# Autodesk Inventor assembly: mobile_robot
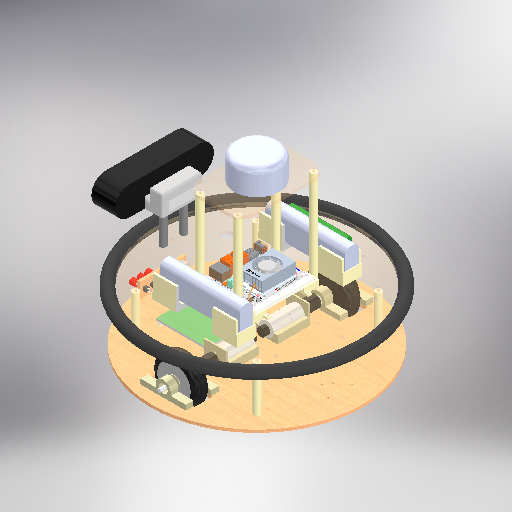
[picture p0: Inventor's stored thumbnail of the model, 512x512]
Saved by Autodesk Inventor 2026 (Build 300175050, 175E)
## iProperties
Created: 2025-06-04
Part Number: mobile_robot
Document SubType Name: Assembly
Designer: satom
Author: satom
## Documents named in this file (32)
- C:\Users\satom\Desktop\Robot\CAD\Inventor\mobile_robot_short.iam
- C:\Users\satom\Desktop\Robot\CAD\Inventor\C - Chassis\layer1.ipt
- C:\Users\satom\Desktop\Robot\CAD\Inventor\D - DriveTrain\wheel_bearing.ipt
- C:\Users\satom\Desktop\Robot\CAD\Inventor\D - DriveTrain\wheel_mount.ipt
- C:\Users\satom\Desktop\Robot\CAD\Inventor\D - DriveTrain\motor_holder.ipt
- C:\Users\satom\Desktop\Robot\CAD\Inventor\solidworks\D - DriveTrain\ball_caster\ball_caster\ball_caster.ipt
- C:\Users\satom\Desktop\Robot\CAD\Inventor\solidworks\D - DriveTrain\motor\motor\motor.ipt
- C:\Users\satom\Desktop\Robot\CAD\Inventor\solidworks\D - DriveTrain\wheel\wheel\wheel.ipt
- C:\Users\satom\Desktop\Robot\CAD\Inventor\solidworks\D - DriveTrain\drive_shaft\drive_shaft\drive_shaft.ipt
- C:\Users\satom\Desktop\Robot\CAD\Inventor\solidworks\D - DriveTrain\ball_bearing\ball_bearing\ball_bearing.ipt
- C:\Users\satom\Desktop\Robot\CAD\Inventor\solidworks\D - DriveTrain\shaft_coupler 6 mm\shaft_coupler 6 mm\shaft_coupler 6 mm.ipt
- C:\Users\satom\Desktop\Robot\CAD\Inventor\solidworks\E - Electronics\Main Board\Main Board\Main Board.ipt
- C:\Users\satom\Desktop\Robot\CAD\Inventor\E - Electronics\1-4_inch_standoff.ipt
- C:\Users\satom\Desktop\Robot\CAD\Inventor\C - Chassis\3inch_standoff.ipt
- C:\Users\satom\Desktop\Robot\CAD\Inventor\C - Chassis\control_panel.ipt
- C:\Users\satom\Desktop\Robot\CAD\Inventor\E - Electronics\status_LED\status_LED\status_LED.ipt
- C:\Users\satom\Desktop\Robot\CAD\Inventor\E - Electronics\rocker_switch\rocker_switch\rocker_switch.ipt
- C:\Users\satom\Desktop\Robot\CAD\Inventor\E - Electronics\button\button\button.ipt
- C:\Users\satom\Desktop\Robot\CAD\Inventor\solidworks\E - Electronics\NiMH_battery\NiMH_battery\NiMH_battery.ipt
- C:\Users\satom\Desktop\Robot\CAD\Inventor\E - Electronics\NiMH_Holder_Front.ipt
- C:\Users\satom\Desktop\Robot\CAD\Inventor\E - Electronics\NiMH_Holder_Back.ipt
- C:\Users\satom\Desktop\Robot\CAD\Inventor\solidworks\E - Electronics\Lion_5V\Lion_5V\Lion_5V.ipt
- C:\Users\satom\Desktop\Robot\CAD\Inventor\E - Electronics\jetson_orin_nano_holder_corner_1.ipt
- C:\Users\satom\Desktop\Robot\CAD\Inventor\E - Electronics\jetson_orin_nano_holder_corner_2.ipt
- C:\Users\satom\Desktop\Robot\CAD\Inventor\E - Electronics\orin_nano\orin_nano\orin_nano.ipt
- C:\Users\satom\Desktop\Robot\CAD\Inventor\C - Chassis\layer2_short.ipt
- C:\Users\satom\Desktop\Robot\CAD\Inventor\C - Chassis\foam_bumper_circular.ipt
- C:\Users\satom\Desktop\Robot\CAD\Inventor\C - Chassis\LiDAR_plate.ipt
- C:\Users\satom\Desktop\Robot\CAD\Inventor\E - Electronics\astra_camera.ipt
- C:\Users\satom\Desktop\Robot\CAD\Inventor\E - Electronics\astra_holder.ipt
- C:\Users\satom\Desktop\Robot\CAD\Inventor\solidworks\E - Electronics\A2_LIDAR\A2_LIDAR\A2_LIDAR.ipt
- C:\Users\satom\Desktop\Robot\CAD\Inventor\C - Chassis\6inch_standoff.ipt
## Components (62 placed, 31 different names)
1. layer1:1 — Mate:1, Mate:2, Mate:3, Mate:4, Mate:5, Mate:6, Mate:7, Mate:8, Mate:9, Mate:10, Mate:11, Mate:12, Mate:13, Mate:14, Mate:15, Mate:16, Mate:17, Mate:18, Mate:19, Mate:20, Mate:21, Mate:22, Mate:23, Mate:56, Mate:57, Mate:66, Mate:67, Mate:68, Mate:69, Mate:70, Mate:71, Mate:72, Mate:73, Mate:74, Mate:75, Mate:76, Flush:3, Mate:88, Mate:89
2. wheel_bearing:1 — Mate:7, Mate:8, Mate:16, Mate:40, Mate:41
3. wheel_mount:1 — Mate:32, Mate:33, Flush:2
4. motor_holder:1 — Mate:2, Mate:3, Mate:26, Mate:27, Mate:56, Mate:57
5. wheel_bearing:2 — Mate:9, Mate:10, Mate:14, Mate:15, Mate:46, Mate:47
6. wheel_mount:2 — Mate:28, Mate:29, Flush:1, Mate:36, Mate:37
7. motor_holder:2 — Mate:1, Mate:4, Mate:24, Mate:25
8. wheel_bearing:3 — Mate:11, Mate:12, Mate:13, Mate:44, Mate:45
9. wheel_mount:3 — Mate:30, Mate:31, Flush:1
10. wheel_bearing:4 — Mate:5, Mate:6, Mate:17, Mate:42, Mate:43
11. wheel_mount:4 — Mate:34, Mate:35, Flush:2, Mate:38, Mate:39
12. ball_caster:1 — Mate:19, Mate:22, Mate:23
13. ball_caster:2 — Mate:18, Mate:20, Mate:21
14. motor:1 — Mate:24, Mate:25, Mate:48, Mate:51
15. motor:2 — Mate:26, Mate:27, Mate:52, Mate:55
16. wheel:1 — Mate:32, Mate:33, Mate:34, Mate:35
17. wheel:2 — Mate:28, Mate:29, Mate:30, Mate:31
18. drive_shaft:1 — Mate:38, Mate:39, Mate:49, Mate:50
19. drive_shaft:2 — Mate:36, Mate:37, Mate:53, Mate:54
20. ball_bearing:1 — Mate:42, Mate:43
21. ball_bearing:2 — Mate:40, Mate:41
22. ball_bearing:3 — Mate:44, Mate:45, Mate:49
23. ball_bearing:4 — Mate:46, Mate:47
24. shaft_coupler 6 mm:1 — Mate:48, Mate:50, Mate:51
25. shaft_coupler 6 mm:2 — Mate:52, Mate:53, Mate:54, Mate:55
26. Main Board:1 — Mate:61, Mate:62, Mate:63, Mate:64, Mate:65
27. 1-4_inch_standoff:1 — Mate:62, Mate:65
28. 1-4_inch_standoff:2 — Mate:63, Mate:64, Mate:66, Mate:67
29. 1-4_inch_standoff:3 — Mate:61, Mate:68
30. 1-4_inch_standoff:4
31. 3inch_standoff:1 — Mate:69, Mate:71
32. 3inch_standoff:2 — Mate:70, Mate:72, Mate:132
33. 3inch_standoff:3 — Mate:73, Mate:74
34. 3inch_standoff:4 — Mate:75, Mate:76, Mate:130, Mate:131
35. control_panel:1 — Flush:3, Mate:88, Mate:89
36. status_LED:1
37. rocker_switch:1
38. button:1
39. button:2
40. button:3
41. NiMH_battery:1 — Mate:135
42. NiMH_battery:2 — Mate:147
43. NiMH_Holder_Front:1 — Mate:134, Mate:138, Mate:139
44. NiMH_Holder_Back:1 — Mate:133, Mate:135, Mate:136, Mate:137
45. NiMH_Holder_Back:2 — Mate:141, Mate:142, Mate:143, Mate:147
46. NiMH_Holder_Front:2 — Mate:144, Mate:145, Mate:146, Mate:148, Flush:151
47. Lion_5V:1 — Mate:148, Flush:151, Mate:149
48. jetson_orin_nano_holder_corner_1:1 — Mate:154, Mate:155
49. jetson_orin_nano_holder_corner_1:2 — Mate:129, Mate:150, Mate:151
50. jetson_orin_nano_holder_corner_2:1 — Mate:156, Mate:157
51. jetson_orin_nano_holder_corner_2:2 — Mate:152, Mate:153
52. orin_nano:1 — Mate:129
53. layer2_short:1 — Mate:130, Mate:131, Mate:132, Mate:133, Mate:134, Mate:136, Mate:137, Mate:138, Mate:139, Mate:141, Mate:142, Mate:143, Mate:144, Mate:145, Mate:146, Mate:149, Mate:150, Mate:151, Mate:152, Mate:153, Mate:154, Mate:155, Mate:156, Mate:157, Mate:158, Mate:159, Mate:164, Mate:165, Mate:166, Mate:168, Mate:169, Mate:170, Mate:171, Mate:178, Mate:179
54. foam_bumper_circular:1 — Mate:158, Mate:159
55. LiDAR_plate:1 — Mate:160, Mate:161, Mate:162, Mate:172, Mate:173, Mate:174, Mate:175, Mate:176, Mate:177
56. astra_camera:1 — Mate:163, Flush:152, Mate:167
57. astra_holder:1 — Mate:163, Mate:164, Mate:165, Mate:166, Flush:152, Mate:167
58. A2_LIDAR:1 — Mate:160, Mate:161, Mate:162
59. 6inch_standoff:1 — Mate:171, Mate:176
60. 6inch_standoff:2 — Mate:168, Mate:174, Mate:175, Mate:179
61. 6inch_standoff:3 — Mate:169, Mate:177, Mate:178
62. 6inch_standoff:4 — Mate:170, Mate:172, Mate:173
## Relationships (149: Mate 144, Flush 5)
- Mate:1: layer1:1 ↔ motor_holder:2
- Mate:2: layer1:1 ↔ motor_holder:1
- Mate:3: layer1:1 ↔ motor_holder:1
- Mate:4: layer1:1 ↔ motor_holder:2
- Mate:5: layer1:1 ↔ wheel_bearing:4
- Mate:6: layer1:1 ↔ wheel_bearing:4
- Mate:7: layer1:1 ↔ wheel_bearing:1
- Mate:8: layer1:1 ↔ wheel_bearing:1
- Mate:9: layer1:1 ↔ wheel_bearing:2
- Mate:10: layer1:1 ↔ wheel_bearing:2
- Mate:11: layer1:1 ↔ wheel_bearing:3
- Mate:12: layer1:1 ↔ wheel_bearing:3
- Mate:13: layer1:1 ↔ wheel_bearing:3
- Mate:14: layer1:1 ↔ wheel_bearing:2
- Mate:15: layer1:1 ↔ wheel_bearing:2
- Mate:16: layer1:1 ↔ wheel_bearing:1
- Mate:17: layer1:1 ↔ wheel_bearing:4
- Mate:18: layer1:1 ↔ ball_caster:2
- Mate:19: layer1:1 ↔ ball_caster:1
- Mate:20: layer1:1 ↔ ball_caster:2
- Mate:21: layer1:1 ↔ ball_caster:2
- Mate:22: layer1:1 ↔ ball_caster:1
- Mate:23: layer1:1 ↔ ball_caster:1
- Mate:24: motor_holder:2 ↔ motor:1
- Mate:25: motor_holder:2 ↔ motor:1
- Mate:26: motor_holder:1 ↔ motor:2
- Mate:27: motor_holder:1 ↔ motor:2
- Mate:28: wheel_mount:2 ↔ wheel:2
- Mate:29: wheel_mount:2 ↔ wheel:2
- Mate:30: wheel_mount:3 ↔ wheel:2
- Mate:31: wheel_mount:3 ↔ wheel:2
- Flush:1: wheel_mount:2 ↔ wheel_mount:3
- Mate:32: wheel_mount:1 ↔ wheel:1
- Mate:33: wheel_mount:1 ↔ wheel:1
- Mate:34: wheel_mount:4 ↔ wheel:1
- Mate:35: wheel_mount:4 ↔ wheel:1
- Flush:2: wheel_mount:1 ↔ wheel_mount:4
- Mate:36: wheel_mount:2 ↔ drive_shaft:2
- Mate:37: wheel_mount:2 ↔ drive_shaft:2
- Mate:38: wheel_mount:4 ↔ drive_shaft:1
- Mate:39: wheel_mount:4 ↔ drive_shaft:1
- Mate:40: wheel_bearing:1 ↔ ball_bearing:2
- Mate:41: wheel_bearing:1 ↔ ball_bearing:2
- Mate:42: wheel_bearing:4 ↔ ball_bearing:1
- Mate:43: wheel_bearing:4 ↔ ball_bearing:1
- Mate:44: wheel_bearing:3 ↔ ball_bearing:3
- Mate:45: wheel_bearing:3 ↔ ball_bearing:3
- Mate:46: wheel_bearing:2 ↔ ball_bearing:4
- Mate:47: wheel_bearing:2 ↔ ball_bearing:4
- Mate:48: motor:1 ↔ shaft_coupler 6 mm:1
- Mate:49: drive_shaft:1 ↔ ball_bearing:3
- Mate:50: drive_shaft:1 ↔ shaft_coupler 6 mm:1
- Mate:51 (3.175 mm): motor:1 ↔ shaft_coupler 6 mm:1
- Mate:52: motor:2 ↔ shaft_coupler 6 mm:2
- Mate:53: drive_shaft:2 ↔ shaft_coupler 6 mm:2
- Mate:54: drive_shaft:2 ↔ shaft_coupler 6 mm:2
- Mate:55 (3.175 mm): motor:2 ↔ shaft_coupler 6 mm:2
- Mate:56: layer1:1 ↔ motor_holder:1
- Mate:57: layer1:1 ↔ motor_holder:1
- [Mate]: Main Board:1 ↔ 1-4_inch_standoff:4
- [Mate]: Main Board:1 ↔ 1-4_inch_standoff:3
- [Mate]: Main Board:1 ↔ 1-4_inch_standoff:4
- Mate:61: Main Board:1 ↔ 1-4_inch_standoff:3
- Mate:62: Main Board:1 ↔ 1-4_inch_standoff:1
- Mate:63: Main Board:1 ↔ 1-4_inch_standoff:2
- Mate:64: Main Board:1 ↔ 1-4_inch_standoff:2
- Mate:65: Main Board:1 ↔ 1-4_inch_standoff:1
- Mate:66: layer1:1 ↔ 1-4_inch_standoff:2
- Mate:67: layer1:1 ↔ 1-4_inch_standoff:2
- Mate:68: layer1:1 ↔ 1-4_inch_standoff:3
- Mate:69: layer1:1 ↔ 3inch_standoff:1
- Mate:70: layer1:1 ↔ 3inch_standoff:2
- Mate:71: layer1:1 ↔ 3inch_standoff:1
- Mate:72: layer1:1 ↔ 3inch_standoff:2
- Mate:73: layer1:1 ↔ 3inch_standoff:3
- Mate:74: layer1:1 ↔ 3inch_standoff:3
- Mate:75: layer1:1 ↔ 3inch_standoff:4
- Mate:76: layer1:1 ↔ 3inch_standoff:4
- [Mate]: control_panel:1 ↔ status_LED:1
- [Mate]: control_panel:1 ↔ status_LED:1
- [Mate]: control_panel:1 ↔ rocker_switch:1
- [Mate]: control_panel:1 ↔ rocker_switch:1
- [Mate]: control_panel:1 ↔ rocker_switch:1
- [Mate]: control_panel:1 ↔ button:1
- [Mate]: control_panel:1 ↔ button:1
- [Mate]: control_panel:1 ↔ button:3
- [Mate]: control_panel:1 ↔ button:2
- [Mate]: control_panel:1 ↔ button:2
- [Mate]: control_panel:1 ↔ button:3
- Flush:3: layer1:1 ↔ control_panel:1
- Mate:88: layer1:1 ↔ control_panel:1
- Mate:89: layer1:1 ↔ control_panel:1
- [Mate]: NiMH_battery:1 ↔ NiMH_Holder_Front:1
- [Mate]: NiMH_battery:1 ↔ NiMH_Holder_Back:1
- [Mate]: NiMH_battery:2 ↔ NiMH_Holder_Back:2
- [Mate]: jetson_orin_nano_holder_corner_2:2 ↔ orin_nano:1
- [Mate]: jetson_orin_nano_holder_corner_1:2 ↔ orin_nano:1
- Mate:129: jetson_orin_nano_holder_corner_1:2 ↔ orin_nano:1
- Mate:130: 3inch_standoff:4 ↔ layer2_short:1
- Mate:131: 3inch_standoff:4 ↔ layer2_short:1
- Mate:132: 3inch_standoff:2 ↔ layer2_short:1
- Mate:133: NiMH_Holder_Back:1 ↔ layer2_short:1
- Mate:134: NiMH_Holder_Front:1 ↔ layer2_short:1
- Mate:135: NiMH_battery:1 ↔ NiMH_Holder_Back:1
- Mate:136: NiMH_Holder_Back:1 ↔ layer2_short:1
- Mate:137: NiMH_Holder_Back:1 ↔ layer2_short:1
- Mate:138: NiMH_Holder_Front:1 ↔ layer2_short:1
- Mate:139: NiMH_Holder_Front:1 ↔ layer2_short:1
- Mate:141: NiMH_Holder_Back:2 ↔ layer2_short:1
- Mate:142: NiMH_Holder_Back:2 ↔ layer2_short:1
- Mate:143: NiMH_Holder_Back:2 ↔ layer2_short:1
- Mate:144: NiMH_Holder_Front:2 ↔ layer2_short:1
- Mate:145: NiMH_Holder_Front:2 ↔ layer2_short:1
- Mate:146: NiMH_Holder_Front:2 ↔ layer2_short:1
- Mate:147: NiMH_battery:2 ↔ NiMH_Holder_Back:2
- Mate:148: NiMH_Holder_Front:2 ↔ Lion_5V:1
- Flush:151: NiMH_Holder_Front:2 ↔ Lion_5V:1
- Mate:149: Lion_5V:1 ↔ layer2_short:1
- Mate:150: jetson_orin_nano_holder_corner_1:2 ↔ layer2_short:1
- Mate:151: jetson_orin_nano_holder_corner_1:2 ↔ layer2_short:1
- Mate:152: jetson_orin_nano_holder_corner_2:2 ↔ layer2_short:1
- Mate:153: jetson_orin_nano_holder_corner_2:2 ↔ layer2_short:1
- Mate:154: jetson_orin_nano_holder_corner_1:1 ↔ layer2_short:1
- Mate:155: jetson_orin_nano_holder_corner_1:1 ↔ layer2_short:1
- Mate:156: jetson_orin_nano_holder_corner_2:1 ↔ layer2_short:1
- Mate:157: jetson_orin_nano_holder_corner_2:1 ↔ layer2_short:1
- Mate:158: layer2_short:1 ↔ foam_bumper_circular:1
- Mate:159: layer2_short:1 ↔ foam_bumper_circular:1
- Mate:160: LiDAR_plate:1 ↔ A2_LIDAR:1
- Mate:161: LiDAR_plate:1 ↔ A2_LIDAR:1
- Mate:162: LiDAR_plate:1 ↔ A2_LIDAR:1
- Mate:163: astra_camera:1 ↔ astra_holder:1
- Mate:164: layer2_short:1 ↔ astra_holder:1
- Mate:165: layer2_short:1 ↔ astra_holder:1
- Mate:166: layer2_short:1 ↔ astra_holder:1
- Flush:152 (-12.7 mm): astra_camera:1 ↔ astra_holder:1
- Mate:167 (25.4 mm): astra_camera:1 ↔ astra_holder:1
- Mate:168: layer2_short:1 ↔ 6inch_standoff:2
- Mate:169: layer2_short:1 ↔ 6inch_standoff:3
- Mate:170: layer2_short:1 ↔ 6inch_standoff:4
- Mate:171: layer2_short:1 ↔ 6inch_standoff:1
- Mate:172: LiDAR_plate:1 ↔ 6inch_standoff:4
- Mate:173: LiDAR_plate:1 ↔ 6inch_standoff:4
- Mate:174: LiDAR_plate:1 ↔ 6inch_standoff:2
- Mate:175: LiDAR_plate:1 ↔ 6inch_standoff:2
- Mate:176: LiDAR_plate:1 ↔ 6inch_standoff:1
- Mate:177: LiDAR_plate:1 ↔ 6inch_standoff:3
- Mate:178: layer2_short:1 ↔ 6inch_standoff:3
- Mate:179: layer2_short:1 ↔ 6inch_standoff:2
